# Autodesk Inventor assembly: 手首関節
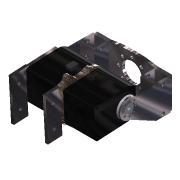
[picture p0: Inventor's stored thumbnail of the model, 180x180]
Saved by Autodesk Inventor 2019.4 (Build 234330000, 330)
## iProperties
Created: 2019-06-16
Part Number: 手首関節
Material: 一般
Document SubType Name: Assembly
Designer: 長谷川翔一
Author: 長谷川翔一
## Documents named in this file (9)
- E:\ロボ研\キャチロボ\キャチロボ2019\CADdata\アーム2019\Wrist\手首関節.iam
- E:\ロボ研\キャチロボ\キャチロボ2019\CADdata\アーム2019\Wrist\KRS-4034HV.ipt
- E:\ロボ研\キャチロボ\キャチロボ2019\CADdata\アーム2019\Wrist\デュアルサーボつなぎフレーム_ポリカ_t3.ipt
- E:\ロボ研\キャチロボ\キャチロボ2019\CADdata\アーム2019\Wrist\ローハイトサーボホーン 2500.ipt
- E:\ロボ研\キャチロボ\キャチロボ2019\CADdata\アーム2019\Wrist\デュアルサーボつなぎフレーム_アルミ(A2017)_t3.ipt
- E:\ロボ研\キャチロボ\キャチロボ2019\CADdata\アーム2019\Wrist\サーボ支え板A_アルミ(A2017)_t1.5.ipt
- E:\ロボ研\キャチロボ\キャチロボ2019\CADdata\アーム2019\Wrist\支え角柱(サーボ用).ipt
- E:\ロボ研\キャチロボ\キャチロボ2019\CADdata\アーム2019\Wrist\サーボ支え板B_アルミ(A2017)_t3.ipt
- E:\ロボ研\キャチロボ\キャチロボ2019\CADdata\アーム2019\Wrist\デュアルサーボつなぎフレームB_アルミ(A2017)_t3.ipt
## Components (12 placed, 8 different names)
1. KRS-4034HV:1 — メイト:1, メイト:2, メイト:3, メイト:4, メイト:5, メイト:6, メイト:7, メイト:9
2. デュアルサーボつなぎフレーム_ポリカ_t3:1 — メイト:1, メイト:2, メイト:3, メイト:4, メイト:5, メイト:10, メイト:18
3. ローハイトサーボホーン 2500:1 — メイト:6, メイト:7, メイト:24, メイト:25, メイト:26, メイト:27, メイト:28
4. KRS-4034HV:2 — メイト:9, メイト:10, メイト:11, メイト:12, メイト:13, メイト:14, メイト:15, メイト:16, メイト:17, メイト:44, メイト:45, メイト:46, メイト:47
5. ローハイトサーボホーン 2500:2 — メイト:11, メイト:12, メイト:19, メイト:20, メイト:21, メイト:22, メイト:23
6. デュアルサーボつなぎフレーム_アルミ(A2017)_t3:1 — メイト:13, メイト:14, メイト:15, メイト:16, メイト:17, メイト:18
7. サーボ支え板A_アルミ(A2017)_t1.5:1 — メイト:19, メイト:20, メイト:21, メイト:22, メイト:23, メイト:29, メイト:30, メイト:31, メイト:35, メイト:36
8. サーボ支え板A_アルミ(A2017)_t1.5:2 — メイト:24, メイト:25, メイト:26, メイト:27, メイト:28, メイト:32, メイト:33, メイト:34
9. 支え角柱(サーボ用):1 — メイト:29, メイト:30, メイト:31, メイト:37, メイト:40, メイト:41
10. 支え角柱(サーボ用):2 — メイト:32, メイト:33, メイト:34, メイト:35, メイト:36, メイト:38, メイト:39
11. サーボ支え板B_アルミ(A2017)_t3:1 — メイト:37, メイト:38, メイト:39, メイト:40, メイト:41
12. デュアルサーボつなぎフレームB_アルミ(A2017)_t3:1 — メイト:44, メイト:45, メイト:46, メイト:47
## Relationships (44: Mate 44)
- メイト:1 [Mate]: KRS-4034HV:1 ↔ デュアルサーボつなぎフレーム_ポリカ_t3:1
- メイト:2 [Mate]: KRS-4034HV:1 ↔ デュアルサーボつなぎフレーム_ポリカ_t3:1
- メイト:3 [Mate]: KRS-4034HV:1 ↔ デュアルサーボつなぎフレーム_ポリカ_t3:1
- メイト:4 [Mate]: KRS-4034HV:1 ↔ デュアルサーボつなぎフレーム_ポリカ_t3:1
- メイト:5 [Mate]: KRS-4034HV:1 ↔ デュアルサーボつなぎフレーム_ポリカ_t3:1
- メイト:6 [Mate]: KRS-4034HV:1 ↔ ローハイトサーボホーン 2500:1
- メイト:7 [Mate]: KRS-4034HV:1 ↔ ローハイトサーボホーン 2500:1
- メイト:9 [Mate]: KRS-4034HV:1 ↔ KRS-4034HV:2
- メイト:10 [Mate]: デュアルサーボつなぎフレーム_ポリカ_t3:1 ↔ KRS-4034HV:2
- メイト:11 [Mate]: KRS-4034HV:2 ↔ ローハイトサーボホーン 2500:2
- メイト:12 [Mate]: KRS-4034HV:2 ↔ ローハイトサーボホーン 2500:2
- メイト:13 [Mate]: KRS-4034HV:2 ↔ デュアルサーボつなぎフレーム_アルミ(A2017)_t3:1
- メイト:14 [Mate]: KRS-4034HV:2 ↔ デュアルサーボつなぎフレーム_アルミ(A2017)_t3:1
- メイト:15 [Mate]: KRS-4034HV:2 ↔ デュアルサーボつなぎフレーム_アルミ(A2017)_t3:1
- メイト:16 [Mate]: KRS-4034HV:2 ↔ デュアルサーボつなぎフレーム_アルミ(A2017)_t3:1
- メイト:17 [Mate]: KRS-4034HV:2 ↔ デュアルサーボつなぎフレーム_アルミ(A2017)_t3:1
- メイト:18 [Mate]: デュアルサーボつなぎフレーム_ポリカ_t3:1 ↔ デュアルサーボつなぎフレーム_アルミ(A2017)_t3:1
- メイト:19 [Mate]: ローハイトサーボホーン 2500:2 ↔ サーボ支え板A_アルミ(A2017)_t1.5:1
- メイト:20 [Mate]: ローハイトサーボホーン 2500:2 ↔ サーボ支え板A_アルミ(A2017)_t1.5:1
- メイト:21 [Mate]: ローハイトサーボホーン 2500:2 ↔ サーボ支え板A_アルミ(A2017)_t1.5:1
- メイト:22 [Mate]: ローハイトサーボホーン 2500:2 ↔ サーボ支え板A_アルミ(A2017)_t1.5:1
- メイト:23 [Mate]: ローハイトサーボホーン 2500:2 ↔ サーボ支え板A_アルミ(A2017)_t1.5:1
- メイト:24 [Mate]: ローハイトサーボホーン 2500:1 ↔ サーボ支え板A_アルミ(A2017)_t1.5:2
- メイト:25 [Mate]: ローハイトサーボホーン 2500:1 ↔ サーボ支え板A_アルミ(A2017)_t1.5:2
- メイト:26 [Mate]: ローハイトサーボホーン 2500:1 ↔ サーボ支え板A_アルミ(A2017)_t1.5:2
- メイト:27 [Mate]: ローハイトサーボホーン 2500:1 ↔ サーボ支え板A_アルミ(A2017)_t1.5:2
- メイト:28 [Mate]: ローハイトサーボホーン 2500:1 ↔ サーボ支え板A_アルミ(A2017)_t1.5:2
- メイト:29 [Mate]: サーボ支え板A_アルミ(A2017)_t1.5:1 ↔ 支え角柱(サーボ用):1
- メイト:30 [Mate]: サーボ支え板A_アルミ(A2017)_t1.5:1 ↔ 支え角柱(サーボ用):1
- メイト:31 [Mate]: サーボ支え板A_アルミ(A2017)_t1.5:1 ↔ 支え角柱(サーボ用):1
- メイト:32 [Mate]: サーボ支え板A_アルミ(A2017)_t1.5:2 ↔ 支え角柱(サーボ用):2
- メイト:33 [Mate]: サーボ支え板A_アルミ(A2017)_t1.5:2 ↔ 支え角柱(サーボ用):2
- メイト:34 [Mate]: サーボ支え板A_アルミ(A2017)_t1.5:2 ↔ 支え角柱(サーボ用):2
- メイト:35 [Mate]: サーボ支え板A_アルミ(A2017)_t1.5:1 ↔ 支え角柱(サーボ用):2
- メイト:36 [Mate]: サーボ支え板A_アルミ(A2017)_t1.5:1 ↔ 支え角柱(サーボ用):2
- メイト:37 [Mate]: 支え角柱(サーボ用):1 ↔ サーボ支え板B_アルミ(A2017)_t3:1
- メイト:38 [Mate]: 支え角柱(サーボ用):2 ↔ サーボ支え板B_アルミ(A2017)_t3:1
- メイト:39 [Mate]: 支え角柱(サーボ用):2 ↔ サーボ支え板B_アルミ(A2017)_t3:1
- メイト:40 [Mate]: 支え角柱(サーボ用):1 ↔ サーボ支え板B_アルミ(A2017)_t3:1
- メイト:41 [Mate]: 支え角柱(サーボ用):1 ↔ サーボ支え板B_アルミ(A2017)_t3:1
- メイト:44 [Mate]: KRS-4034HV:2 ↔ デュアルサーボつなぎフレームB_アルミ(A2017)_t3:1
- メイト:45 [Mate]: KRS-4034HV:2 ↔ デュアルサーボつなぎフレームB_アルミ(A2017)_t3:1
- メイト:46 [Mate]: KRS-4034HV:2 ↔ デュアルサーボつなぎフレームB_アルミ(A2017)_t3:1
- メイト:47 [Mate]: KRS-4034HV:2 ↔ デュアルサーボつなぎフレームB_アルミ(A2017)_t3:1
